# Autodesk Inventor assembly: LauncherFrame
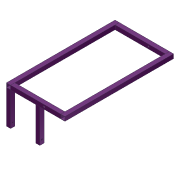
[picture p0: Inventor's stored thumbnail of the model, 180x180]
Saved by Autodesk Inventor 2012 (Build 160160000, 160)
## iProperties
Created: 2013-01-22
Part Number: LauncherFrame
Document SubType Name: Assembly
Designer: JesseK
Mass: 955.115 g
Surface Area: 4462.15 cm^2
Volume: 352.441 cm^3
Density: 2.71 g/cm^3
Author: JesseK
## Documents named in this file (4)
- Z:\UserData\Documents\Inventor\team1885frc\Robot2013\LauncherRearrange\LauncherFrame.iam
- Z:\UserData\Documents\Inventor\team1885frc\Robot2013\LauncherRearrange\CrossFrameRail.ipt
- Z:\UserData\Documents\Inventor\team1885frc\Robot2013\LauncherRearrange\FrontRearRail.ipt
- Z:\UserData\Documents\Inventor\team1885frc\Robot2013\LauncherRearrange\VerticalConveyorSupport.ipt
## Components (6 placed, 3 different names)
1. CrossFrameRail:1 — Flush:3, Flush:4, Mate:5
2. CrossFrameRail:2 — Mate:1, Flush:1, Mate:2, Flush:2, Mate:3, Mate:4, Mate:7, Mate:9, Mate:10
3. FrontRearRail:1 — Mate:1, Flush:1, Mate:3, Mate:6, Mate:11
4. FrontRearRail:2 — Mate:2, Flush:2, Mate:4, Flush:3, Flush:4, Mate:5
5. VerticalConveyorSupport:1 — Mate:6, Mate:11, Mate:14
6. VerticalConveyorSupport:2 — Mate:7, Mate:9, Mate:10, Mate:14
## Relationships (15: Mate 11, Flush 4)
- Mate:1: CrossFrameRail:2 ↔ FrontRearRail:1
- Flush:1: CrossFrameRail:2 ↔ FrontRearRail:1
- Mate:2: CrossFrameRail:2 ↔ FrontRearRail:2
- Flush:2: CrossFrameRail:2 ↔ FrontRearRail:2
- Mate:3: CrossFrameRail:2 ↔ FrontRearRail:1
- Mate:4: CrossFrameRail:2 ↔ FrontRearRail:2
- Flush:3: CrossFrameRail:1 ↔ FrontRearRail:2
- Flush:4: CrossFrameRail:1 ↔ FrontRearRail:2
- Mate:5: CrossFrameRail:1 ↔ FrontRearRail:2
- Mate:6: FrontRearRail:1 ↔ VerticalConveyorSupport:1
- Mate:7: CrossFrameRail:2 ↔ VerticalConveyorSupport:2
- Mate:9: CrossFrameRail:2 ↔ VerticalConveyorSupport:2
- Mate:10: CrossFrameRail:2 ↔ VerticalConveyorSupport:2
- Mate:11: FrontRearRail:1 ↔ VerticalConveyorSupport:1
- Mate:14 (152.4 mm): VerticalConveyorSupport:1 ↔ VerticalConveyorSupport:2
